# Autodesk Inventor assembly: g16
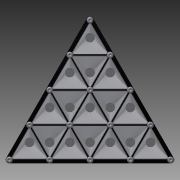
[picture p0: Inventor's stored thumbnail of the model, 180x180]
Saved by Autodesk Inventor 2013 (Build 170138000, 138)
## iProperties
Created: 2013-03-21
Part Number: g16
Document SubType Name: Assembly
Designer: TechShop Member
Author: TechShop Member
## Documents named in this file (11)
- Z:\beth On My Mac\Dropbox\art\2013\03mar\grid16_rev2\g16.iam
- Z:\beth On My Mac\Dropbox\art\2013\03mar\grid16_rev2\g16-bezel.ipt
- Z:\beth On My Mac\Dropbox\art\2013\03mar\grid16_rev2\g16-pixel.ipt
- Z:\beth On My Mac\Dropbox\art\2013\03mar\grid16_rev2\g16-retainer.ipt
- \\vmware-host\Shared Folders\Documents\Inventor\Content Center Files\R2013\en-US\ANSI B18.3.4M(2)\ANSI B18.3.4M - M3 x 0.5 x 30(1).ipt
- Z:\beth On My Mac\Dropbox\art\2013\03mar\grid16_rev2\g16-ledframe.ipt
- Z:\beth On My Mac\Dropbox\art\2013\03mar\grid16_rev2\g16-ledbase.ipt
- Z:\beth On My Mac\Dropbox\art\2013\03mar\grid16_rev2\g16-strut1.ipt
- Z:\beth On My Mac\Dropbox\art\2013\03mar\grid16_rev2\g16-strut2.ipt
- Z:\beth On My Mac\Dropbox\art\2013\03mar\grid16_rev2\g16-baseplate.ipt
- Z:\beth On My Mac\Dropbox\art\2013\03mar\grid16_rev2\g16-reflector.ipt
## Components (39 placed, 10 different names)
1. g16-bezel:1 — Mate:1, Insert:1, Insert:2, Insert:3, Insert:4, Insert:5, Insert:6, Insert:7, Insert:8, Insert:9, Insert:10, Insert:11, Insert:12, Insert:13, Insert:14, Insert:15, Insert:16, Insert:17, Insert:18, Insert:19, Insert:20, Insert:21, Insert:22, Insert:23, Insert:24, Insert:25, Insert:26, Insert:27, Insert:28, Insert:29, Insert:30, Insert:31, Insert:32, Mate:2, Mate:3, Insert:33, Insert:34, Insert:35, Insert:36, Insert:37, Insert:38, Insert:39, Insert:40, Insert:41, Insert:42, Insert:43, Insert:44, Insert:45, Insert:46, Insert:47
2. g16-retainer:1 — Mate:2, Mate:3, Mate:12, Mate:13
3. g16-reflector:1 — Mate:12, Mate:13, Mate:14, Mate:15
4. Forged Hexagon Socket Button Head Cap Screw - Metric M3 x 0.5 x 30:1 — Insert:33
5. Forged Hexagon Socket Button Head Cap Screw - Metric M3 x 0.5 x 30:2 — Insert:34
6. Forged Hexagon Socket Button Head Cap Screw - Metric M3 x 0.5 x 30:3 — Insert:35
7. Forged Hexagon Socket Button Head Cap Screw - Metric M3 x 0.5 x 30:4 — Insert:36
8. Forged Hexagon Socket Button Head Cap Screw - Metric M3 x 0.5 x 30:5 — Insert:37
9. Forged Hexagon Socket Button Head Cap Screw - Metric M3 x 0.5 x 30:6 — Insert:38
10. Forged Hexagon Socket Button Head Cap Screw - Metric M3 x 0.5 x 30:7 — Insert:39
11. Forged Hexagon Socket Button Head Cap Screw - Metric M3 x 0.5 x 30:8 — Insert:40
12. Forged Hexagon Socket Button Head Cap Screw - Metric M3 x 0.5 x 30:9 — Insert:41
13. Forged Hexagon Socket Button Head Cap Screw - Metric M3 x 0.5 x 30:10 — Insert:42
14. Forged Hexagon Socket Button Head Cap Screw - Metric M3 x 0.5 x 30:11 — Insert:43
15. Forged Hexagon Socket Button Head Cap Screw - Metric M3 x 0.5 x 30:12 — Insert:44
16. Forged Hexagon Socket Button Head Cap Screw - Metric M3 x 0.5 x 30:13 — Insert:45
17. Forged Hexagon Socket Button Head Cap Screw - Metric M3 x 0.5 x 30:14 — Insert:46
18. Forged Hexagon Socket Button Head Cap Screw - Metric M3 x 0.5 x 30:15 — Insert:47
19. g16-pixel:1 — Mate:1, Insert:1, Insert:22
20. g16-pixel:2 — Insert:2, Insert:3
21. g16-pixel:3 — Insert:4, Insert:24
22. g16-pixel:4 — Insert:5, Insert:27
23. g16-pixel:5 — Insert:16, Insert:31
24. g16-pixel:6 — Insert:10, Insert:23
25. g16-pixel:7 — Insert:13, Insert:21
26. g16-pixel:8 — Insert:12, Insert:29
27. g16-pixel:9 — Insert:14, Insert:30
28. g16-pixel:10 — Insert:7, Insert:25
29. g16-pixel:11 — Insert:15, Insert:20
30. g16-pixel:12 — Insert:11, Insert:19
31. g16-pixel:13 — Insert:9, Insert:28
32. g16-pixel:14 — Insert:6, Insert:26
33. g16-pixel:15 — Insert:8, Insert:18
34. g16-pixel:16 — Insert:17, Insert:32
35. g16-ledframe:1 — Mate:4, Mate:5, Mate:14, Mate:15
36. g16-ledbase:1 — Mate:4, Mate:5, Mate:6, Mate:7, Mate:8, Mate:9
37. g16-strut1:1 — Mate:6, Mate:7, Mate:10, Mate:11
38. g16-strut2:1 — Mate:8, Mate:9
39. g16-baseplate:1 — Mate:10, Mate:11
## Relationships (62: Insert 47, Mate 15)
- Mate:1: g16-bezel:1 ↔ g16-pixel:1
- Insert:1: g16-bezel:1 ↔ g16-pixel:1
- Insert:2: g16-bezel:1 ↔ g16-pixel:2
- Insert:3: g16-bezel:1 ↔ g16-pixel:2
- Insert:4: g16-bezel:1 ↔ g16-pixel:3
- Insert:5: g16-bezel:1 ↔ g16-pixel:4
- Insert:6: g16-bezel:1 ↔ g16-pixel:14
- Insert:7: g16-bezel:1 ↔ g16-pixel:10
- Insert:8: g16-bezel:1 ↔ g16-pixel:15
- Insert:9: g16-bezel:1 ↔ g16-pixel:13
- Insert:10: g16-bezel:1 ↔ g16-pixel:6
- Insert:11: g16-bezel:1 ↔ g16-pixel:12
- Insert:12: g16-bezel:1 ↔ g16-pixel:8
- Insert:13: g16-bezel:1 ↔ g16-pixel:7
- Insert:14: g16-bezel:1 ↔ g16-pixel:9
- Insert:15: g16-bezel:1 ↔ g16-pixel:11
- Insert:16: g16-bezel:1 ↔ g16-pixel:5
- Insert:17: g16-bezel:1 ↔ g16-pixel:16
- Insert:18: g16-bezel:1 ↔ g16-pixel:15
- Insert:19: g16-bezel:1 ↔ g16-pixel:12
- Insert:20: g16-bezel:1 ↔ g16-pixel:11
- Insert:21: g16-bezel:1 ↔ g16-pixel:7
- Insert:22: g16-bezel:1 ↔ g16-pixel:1
- Insert:23: g16-bezel:1 ↔ g16-pixel:6
- Insert:24: g16-bezel:1 ↔ g16-pixel:3
- Insert:25: g16-bezel:1 ↔ g16-pixel:10
- Insert:26: g16-bezel:1 ↔ g16-pixel:14
- Insert:27: g16-bezel:1 ↔ g16-pixel:4
- Insert:28: g16-bezel:1 ↔ g16-pixel:13
- Insert:29: g16-bezel:1 ↔ g16-pixel:8
- Insert:30: g16-bezel:1 ↔ g16-pixel:9
- Insert:31: g16-bezel:1 ↔ g16-pixel:5
- Insert:32: g16-bezel:1 ↔ g16-pixel:16
- Mate:2: g16-bezel:1 ↔ g16-retainer:1
- Mate:3: g16-bezel:1 ↔ g16-retainer:1
- Mate:4: g16-ledframe:1 ↔ g16-ledbase:1
- Mate:5: g16-ledframe:1 ↔ g16-ledbase:1
- Mate:6: g16-ledbase:1 ↔ g16-strut1:1
- Mate:7: g16-ledbase:1 ↔ g16-strut1:1
- Mate:8: g16-ledbase:1 ↔ g16-strut2:1
- Mate:9: g16-ledbase:1 ↔ g16-strut2:1
- Mate:10: g16-strut1:1 ↔ g16-baseplate:1
- Mate:11: g16-strut1:1 ↔ g16-baseplate:1
- Mate:12: g16-retainer:1 ↔ g16-reflector:1
- Mate:13: g16-retainer:1 ↔ g16-reflector:1
- Mate:14: g16-reflector:1 ↔ g16-ledframe:1
- Mate:15: g16-reflector:1 ↔ g16-ledframe:1
- Insert:33: g16-bezel:1 ↔ Forged Hexagon Socket Button Head Cap Screw - Metric M3 x 0.5 x 30:1
- Insert:34: g16-bezel:1 ↔ Forged Hexagon Socket Button Head Cap Screw - Metric M3 x 0.5 x 30:2
- Insert:35: g16-bezel:1 ↔ Forged Hexagon Socket Button Head Cap Screw - Metric M3 x 0.5 x 30:3
- Insert:36: g16-bezel:1 ↔ Forged Hexagon Socket Button Head Cap Screw - Metric M3 x 0.5 x 30:4
- Insert:37: g16-bezel:1 ↔ Forged Hexagon Socket Button Head Cap Screw - Metric M3 x 0.5 x 30:5
- Insert:38: g16-bezel:1 ↔ Forged Hexagon Socket Button Head Cap Screw - Metric M3 x 0.5 x 30:6
- Insert:39: g16-bezel:1 ↔ Forged Hexagon Socket Button Head Cap Screw - Metric M3 x 0.5 x 30:7
- Insert:40: g16-bezel:1 ↔ Forged Hexagon Socket Button Head Cap Screw - Metric M3 x 0.5 x 30:8
- Insert:41: g16-bezel:1 ↔ Forged Hexagon Socket Button Head Cap Screw - Metric M3 x 0.5 x 30:9
- Insert:42: g16-bezel:1 ↔ Forged Hexagon Socket Button Head Cap Screw - Metric M3 x 0.5 x 30:10
- Insert:43: g16-bezel:1 ↔ Forged Hexagon Socket Button Head Cap Screw - Metric M3 x 0.5 x 30:11
- Insert:44: g16-bezel:1 ↔ Forged Hexagon Socket Button Head Cap Screw - Metric M3 x 0.5 x 30:12
- Insert:45: g16-bezel:1 ↔ Forged Hexagon Socket Button Head Cap Screw - Metric M3 x 0.5 x 30:13
- Insert:46: g16-bezel:1 ↔ Forged Hexagon Socket Button Head Cap Screw - Metric M3 x 0.5 x 30:14
- Insert:47: g16-bezel:1 ↔ Forged Hexagon Socket Button Head Cap Screw - Metric M3 x 0.5 x 30:15
